# Autodesk Inventor assembly: New_Case
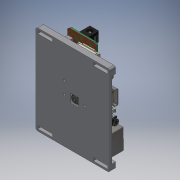
[picture p0: Inventor's stored thumbnail of the model, 180x180]
Saved by Autodesk Inventor 2017 (Build 210142000, 142)
## iProperties
Created: 2017-11-02
Part Number: New_Case
Document SubType Name: Assembly
Designer: P. Baesso
Author: P. Baesso
## Documents named in this file (5)
- C:\Rymapt\ethoscope_hardware\Assembled\New_Case.iam
- C:\Rymapt\ethoscope_hardware\core\RPi3\RPi3_ModelB.ipt
- C:\Rymapt\ethoscope_hardware\core_Rymapt\PiCase\lowerPiCase_small.ipt
- C:\Rymapt\ethoscope_hardware\core\RPi3\RasPi_Camera.ipt
- C:\Rymapt\ethoscope_hardware\Shield\Files\PCB_R2D2.iam
## Components (4 placed, 4 different names)
1. RPi3_ModelB:1 — Angle:1, Angle:2, Flush:1, Flush:2, Mate:4, Flush:3, Mate:5, Flush:4
2. lowerPiCase_small:1 — Mate:1, Mate:2, Mate:3, Angle:1, Angle:2, Flush:1, Flush:2, Mate:4
3. RasPi_Camera:1 — Mate:1, Mate:2, Mate:3
4. PCB_R2D2:1 [sub-assembly] — Flush:3, Mate:5, Flush:4
## Relationships (11: Mate 5, Flush 4, Angle 2)
- Mate:1: lowerPiCase_small:1 ↔ RasPi_Camera:1
- Mate:2: lowerPiCase_small:1 ↔ RasPi_Camera:1
- Mate:3: lowerPiCase_small:1 ↔ RasPi_Camera:1
- Angle:1 (0 deg): RPi3_ModelB:1 ↔ lowerPiCase_small:1
- Angle:2 (0 deg): RPi3_ModelB:1 ↔ lowerPiCase_small:1
- Flush:1 (10.5 mm): RPi3_ModelB:1 ↔ lowerPiCase_small:1
- Flush:2: RPi3_ModelB:1 ↔ lowerPiCase_small:1
- Mate:4: RPi3_ModelB:1 ↔ lowerPiCase_small:1
- Flush:3: RPi3_ModelB:1 ↔ PCB_R2D2:1
- Mate:5 (1 mm): RPi3_ModelB:1 ↔ PCB_R2D2:1
- Flush:4: RPi3_ModelB:1 ↔ PCB_R2D2:1
